# Autodesk Inventor assembly: Ebox_assy
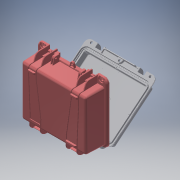
[picture p0: Inventor's stored thumbnail of the model, 180x180]
Saved by Autodesk Inventor 2019.4 (Build 234330000, 330)
## iProperties
Created: 2021-02-08
Part Number: Ebox_assy
Document SubType Name: Assembly
Designer: Jorian Brusind
Author: Jorian Brusind
## Documents named in this file (5)
- C:\Users\Jorian Brusind\Documents\GitHub\PersonalProjects\HyperRail\Inventor Files\Ebox_assy.iam
- C:\Users\Jorian Brusind\Documents\GitHub\PersonalProjects\HyperRail\Inventor Files\se300-t-b.iam
- C:\Users\Jorian Brusind\Documents\GitHub\PersonalProjects\HyperRail\Inventor Files\DM332T_Stepper.ipt
- C:\Users\Jorian Brusind\Documents\GitHub\PersonalProjects\Inventor Projects\S-201-24.ipt
- C:\Users\Jorian Brusind\Documents\GitHub\PersonalProjects\Inventor Projects\Useful models\Raspberry Pi 3.iam
## Components (7 placed, 4 different names)
1. se300-t-b:1 [sub-assembly] — Mate:1, Mate:2, Mate:3, Mate:4, Mate:9, Mate:10, Mate:11, Mate:12, Mate:14, Mate:19
2. DM332T_Stepper:1 — Mate:2, Mate:13, Flush:1, Mate:14, Mate:15
3. DM332T_Stepper:2 — Mate:1, Mate:15, Mate:17
4. DM332T_Stepper:3 — Mate:4, Mate:12, Mate:13, Flush:1, Mate:16, Flush:2
5. DM332T_Stepper:4 — Mate:3, Mate:16, Mate:17, Flush:2
6. S-201-24:1 — Mate:9, Mate:10, Mate:11, Mate:18, Flush:3
7. Raspberry Pi 3:1 [sub-assembly] — Mate:18, Mate:19, Flush:3
## Relationships (18: Mate 15, Flush 3)
- Mate:1: se300-t-b:1 ↔ DM332T_Stepper:2
- Mate:2: se300-t-b:1 ↔ DM332T_Stepper:1
- Mate:3: se300-t-b:1 ↔ DM332T_Stepper:4
- Mate:4: se300-t-b:1 ↔ DM332T_Stepper:3
- Mate:9 (5 mm): se300-t-b:1 ↔ S-201-24:1
- Mate:10: se300-t-b:1 ↔ S-201-24:1
- Mate:11 (5 mm): se300-t-b:1 ↔ S-201-24:1
- Mate:12 (5 mm): se300-t-b:1 ↔ DM332T_Stepper:3
- Mate:13 (5 mm): DM332T_Stepper:1 ↔ DM332T_Stepper:3
- Flush:1: DM332T_Stepper:1 ↔ DM332T_Stepper:3
- Mate:14 (5 mm): se300-t-b:1 ↔ DM332T_Stepper:1
- Mate:15 (5 mm): DM332T_Stepper:1 ↔ DM332T_Stepper:2
- Mate:16 (5 mm): DM332T_Stepper:3 ↔ DM332T_Stepper:4
- Mate:17 (5 mm): DM332T_Stepper:2 ↔ DM332T_Stepper:4
- Flush:2: DM332T_Stepper:3 ↔ DM332T_Stepper:4
- Mate:18 (5 mm): S-201-24:1 ↔ Raspberry Pi 3:1
- Mate:19 (5 mm): se300-t-b:1 ↔ Raspberry Pi 3:1
- Flush:3: S-201-24:1 ↔ Raspberry Pi 3:1
